# Autodesk Inventor assembly: Stackup
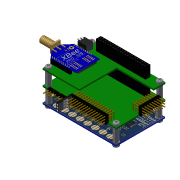
[picture p0: Inventor's stored thumbnail of the model, 180x180]
Saved by Autodesk Inventor 2015 (Build 190159000, 159)
## iProperties
Created: 2014-08-28
Part Number: Stackup
Document SubType Name: Assembly
Designer: david
Author: david
## Documents named in this file (6)
- C:\SharedDrive\Dropbox\ICARUS\Rover\MECHANICAL\810002_ASY-FAST ROVER v2\813006_FAST ROVER v2 CHASSIS ELECTRONICS\Stackup.iam
- C:\SharedDrive\Dropbox\FAST Robotics\Products\811000_Parallax Quickstart\CAD\811000_Parallax Quickstart\811000.iam
- C:\SharedDrive\Dropbox\FAST Robotics\Products\810003_Radio Shield\MECH\810003_Radio Shield\810003A\810003A-XX.iam
- C:\SharedDrive\Dropbox\FAST Robotics\Products\810501_Shield Hardware Kit\CAD\Imported Components\500503\500503.ipt
- C:\SharedDrive\Dropbox\FAST Robotics\Products\810501_Shield Hardware Kit\CAD\Imported Components\500504\500504.ipt
- C:\SharedDrive\Dropbox\FAST Robotics\Products\810501_Shield Hardware Kit\CAD\Imported Components\525501\525501.ipt
## Components (18 placed, 5 different names)
1. 811000:1 [sub-assembly] — Flush:1, Flush:2, Flush:5, Flush:6, Mate:1, Insert:1, Insert:2, Insert:3, Insert:4, Insert:5, Insert:6, Insert:7, Insert:8
2. 811000:2 [sub-assembly] — Flush:1, Flush:2, Flush:3, Flush:4, Insert:9, Insert:10, Insert:11, Insert:12, Mate:2
3. 810003A-XX:1 [sub-assembly] — Flush:3, Flush:4, Insert:13, Insert:14, Insert:15, Mate:3
4. 500503:1 — Insert:1
5. 500504:1 — Insert:14
6. 525501:1 — Insert:5
7. 500503:2 — Insert:3
8. 500503:3 — Insert:4
9. 500503:4 — Insert:2
10. 525501:2 — Insert:6
11. 525501:3 — Insert:7, Mate:2
12. 525501:4 — Insert:8
13. 525501:5 — Insert:11
14. 525501:6 — Insert:10
15. 525501:7 — Insert:9, Mate:3
16. 500504:2 — Insert:15
17. 500504:3 — Insert:13
18. 500504:4 — Insert:12
## Relationships (24: Insert 15, Flush 6, Mate 3)
- Flush:1: 811000:1 ↔ 811000:2
- Flush:2: 811000:1 ↔ 811000:2
- Flush:3: 811000:2 ↔ 810003A-XX:1
- Flush:4: 811000:2 ↔ 810003A-XX:1
- Flush:5: 811000:1
- Flush:6: 811000:1
- Mate:1: 811000:1
- Insert:1: 811000:1 ↔ 500503:1
- Insert:2: 811000:1 ↔ 500503:4
- Insert:3: 811000:1 ↔ 500503:2
- Insert:4: 811000:1 ↔ 500503:3
- Insert:5: 811000:1 ↔ 525501:1
- Insert:6: 811000:1 ↔ 525501:2
- Insert:7: 811000:1 ↔ 525501:3
- Insert:8: 811000:1 ↔ 525501:4
- Insert:9: 811000:2 ↔ 525501:7
- Insert:10: 811000:2 ↔ 525501:6
- Insert:11: 811000:2 ↔ 525501:5
- Insert:12: 811000:2 ↔ 500504:4
- Insert:13: 810003A-XX:1 ↔ 500504:3
- Insert:14: 810003A-XX:1 ↔ 500504:1
- Insert:15: 810003A-XX:1 ↔ 500504:2
- Mate:2: 811000:2 ↔ 525501:3
- Mate:3: 810003A-XX:1 ↔ 525501:7
